# Autodesk Inventor assembly: Assembly cajon
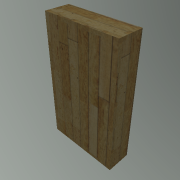
[picture p0: Inventor's stored thumbnail of the model, 180x180]
Saved by Autodesk Inventor 2015 (Build 190159000, 159)
## iProperties
Created: 2016-01-26
Part Number: Assembly cajon
Document SubType Name: Assembly
Designer: iberopuebla
Author: iberopuebla
## Documents named in this file (4)
- H:\3d\Assembly cajon.iam
- H:\3d\cajon abajo.ipt
- H:\3d\cajon front.ipt
- H:\3d\cajon lat.ipt
## Components (5 placed, 3 different names)
1. cajon abajo:1 — Flush:1, Mate:1, Mate:2, Flush:2, Flush:3, Mate:3, Mate:4, Flush:4, Flush:5, Flush:6, Mate:5, Flush:7, Flush:8, Mate:6, Flush:9
2. cajon front:1 — Flush:1, Mate:1, Mate:2, Flush:2
3. cajon lat:1 — Flush:5, Flush:6, Mate:5, Flush:7
4. cajon front:2 — Flush:8, Mate:6, Flush:9
5. cajon lat:2 — Flush:3, Mate:3, Mate:4, Flush:4
## Relationships (15: Flush 9, Mate 6)
- Flush:1: cajon abajo:1 ↔ cajon front:1
- Mate:1: cajon abajo:1 ↔ cajon front:1
- Mate:2: cajon abajo:1 ↔ cajon front:1
- Flush:2: cajon abajo:1 ↔ cajon front:1
- Flush:3: cajon abajo:1 ↔ cajon lat:2
- Mate:3: cajon abajo:1 ↔ cajon lat:2
- Mate:4: cajon abajo:1 ↔ cajon lat:2
- Flush:4: cajon abajo:1 ↔ cajon lat:2
- Flush:5: cajon abajo:1 ↔ cajon lat:1
- Flush:6: cajon abajo:1 ↔ cajon lat:1
- Mate:5: cajon abajo:1 ↔ cajon lat:1
- Flush:7: cajon abajo:1 ↔ cajon lat:1
- Flush:8: cajon abajo:1 ↔ cajon front:2
- Mate:6: cajon abajo:1 ↔ cajon front:2
- Flush:9: cajon abajo:1 ↔ cajon front:2
